# Autodesk Inventor assembly: Bumper
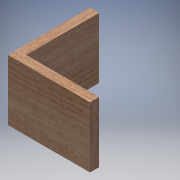
[picture p0: Inventor's stored thumbnail of the model, 180x180]
Saved by Autodesk Inventor 2017 (Build 210142000, 142)
## iProperties
Created: 2017-02-12
Part Number: Bumper
Document SubType Name: Assembly
Designer: kingb
Author: kingb
## Documents named in this file (3)
- C:\Users\kingb\Desktop\CAD\Bumper.iam
- C:\Users\kingb\Desktop\CAD\D1.ipt
- C:\Users\kingb\Desktop\CAD\D2.ipt
## Components (2 placed, 2 different names)
1. D1:1 — Mate:1, Flush:1, Mate:2
2. D2:1 — Mate:1, Flush:1, Mate:2
## Relationships (3: Mate 2, Flush 1)
- Mate:1: D1:1 ↔ D2:1
- Flush:1: D1:1 ↔ D2:1
- Mate:2: D1:1 ↔ D2:1
